# Autodesk Inventor assembly: MSF-25-6-8
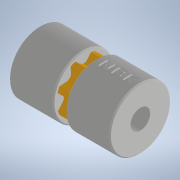
[picture p0: Inventor's stored thumbnail of the model, 180x180]
Saved by Autodesk Inventor 2021 (Build 250183000, 183)
## iProperties
Category: PARTsolutions
Company: NBK
Created: 2026-05-20
Part Number: MSF-25-6-8
Catalog Web Link: www.3dfindit.com
Description: MSF-
Vendor: NBK
Document SubType Name: Assembly
Designer: psAdmin
Manufacturer: NBK
Mass: 16.6411 g
Surface Area: 86.6956 cm^2
Volume: 16.6411 cm^3
Density: 1 g/cm^3
Title: MSF-25-6-8
Author: Cadenas PARTsolutions
PSOL_IDENT_0: {$CADENAS_DATA/23d-libs/nbk/motion_control_parts/couplicon_mini/serration_type/msf_asmtab.prj},176 {
PSOL_IDENT_1: VTYP=3D},{STYP=ASSTAB},{NB=MSF-25-6-8},{LINA=MSF-25-6-8},{NN=MSF},{DATE=08.05.2026 02:12:36},{GEOMDA
PSOL_IDENT_2: TE=29.06.2020 04:55:20},{VERSION=},{LINEID=190},{WBVAR=D1D2},{WBNUMERIC=}  {NB=MSF-25-6-8},{LINA=MSF
PSOL_IDENT_3: -25-6-8},{KT=DUMMY},{CN=MSF-25},{D1D2=6-8},{D1D2X1='6-6','6-6.35','6-8','6-10','6-12','6.35-6.35','6
PSOL_IDENT_4: .35-8','6.35-10','6.35-12','8-8','8-10','8-12','10-10','10-12','12-12'},{A=25},{B=18},{L=12},{W=41},
PSOL_IDENT_5: {F=6},{M=M4},{WT=1.7},{SC=17},{SK=22},{SD=10/10},{PPATH=../msf/msf_asmtpl.prj},{CNSORDERNO=MSF-25-6-
PSOL_IDENT_6: 8}
NB: MSF-25-6-8
NN: MSF
NBSYN: $CN.-$D1D2.
LINA: MSF-25-6-8
CATALOG: NBK (Nabeya Bi-tech Kaisha
CN: MSF-25
D1D2: 6-8
A: 25
B: 18
L: 12
W: 41
F: 6
M: M4
WT: 1.7
SC: 17
SK: 22
SD: 10/10
SUPPLIER: NBK
ARTICLENO: MSF-25-6-8
BOMINFO: MSF-25-6-8
CREATOR: CADENAS GmbH
## Documents named in this file (4)
- e:\temp\worker_COMMON_218\temp\tmp_5544_62_vH4bI\format_0\MSF-25-6-8.iam
- e:\temp\worker_COMMON_218\temp\tmp_5544_62_vH4bI\format_0\MSF-25 - 6-8 Casing 1.ipt
- e:\temp\worker_COMMON_218\temp\tmp_5544_62_vH4bI\format_0\MSF-25 Sleeve.ipt
- e:\temp\worker_COMMON_218\temp\tmp_5544_62_vH4bI\format_0\MSF-25 - 6-8 Casing 2.ipt
## Components (3 placed, 3 different names)
1. MSF-25 - 6-8 Casing 1:1 — left_XY@1 <-> left_XY@2, left_Z@1 <-> left_Z@2, left_YZ@1 <-> left_YZ@2
2. MSF-25 Sleeve:1 — left_XY@1 <-> left_XY@2, left_Z@1 <-> left_Z@2, left_YZ@1 <-> left_YZ@2, right_XY@2 <-> left_XY@3, right_Z@2 <-> left_Z@3, right_YZ@2 <-> left_YZ@3
3. MSF-25 - 6-8 Casing 2:1 — right_XY@2 <-> left_XY@3, right_Z@2 <-> left_Z@3, right_YZ@2 <-> left_YZ@3
## Relationships (6: Mate 3, Angle 2, Flush 1)
- left_XY@1 <-> left_XY@2 [Flush]: MSF-25 - 6-8 Casing 1:1 ↔ MSF-25 Sleeve:1
- left_Z@1 <-> left_Z@2 [Mate]: MSF-25 - 6-8 Casing 1:1 ↔ MSF-25 Sleeve:1
- left_YZ@1 <-> left_YZ@2 [Angle] (0 deg): MSF-25 - 6-8 Casing 1:1 ↔ MSF-25 Sleeve:1
- right_XY@2 <-> left_XY@3 [Mate]: MSF-25 Sleeve:1 ↔ MSF-25 - 6-8 Casing 2:1
- right_Z@2 <-> left_Z@3 [Mate]: MSF-25 Sleeve:1 ↔ MSF-25 - 6-8 Casing 2:1
- right_YZ@2 <-> left_YZ@3 [Angle] (180 deg): MSF-25 Sleeve:1 ↔ MSF-25 - 6-8 Casing 2:1
